# Autodesk Inventor assembly: Front Panel Assembly
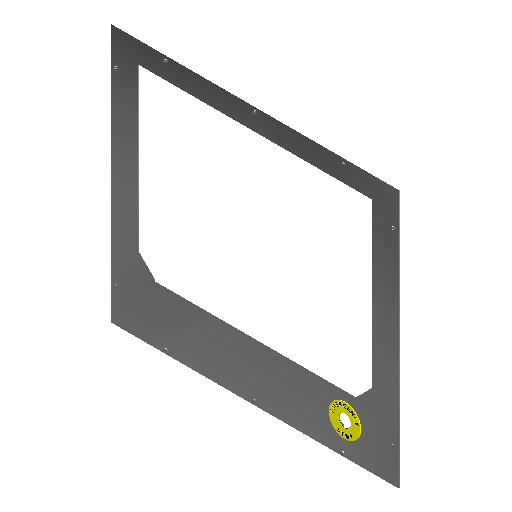
[picture p0: Inventor's stored thumbnail of the model, 512x512]
Saved by Autodesk Inventor 2023.2 (Build 272271000, 271)
## iProperties
Created: 2023-02-06
Part Number: Front Panel Assembly
Document SubType Name: Assembly
Designer: remop
Author: remop
## Documents named in this file (5)
- C:\Users\remop\OneDrive\Documents\Inventor\3D Printers\LuEVO\Mk5_FullKinematic\Front Panel Assembly.iam
- C:\Users\remop\OneDrive\Documents\Inventor\3D Printers\LuEVO\Mk5_FullKinematic\Front Panel.ipt
- C:\Users\remop\OneDrive\Documents\Inventor\Content Center Files\R2023\en-US\AS 1420\AS 1420 - 1973 - M3 x 6.ipt
- C:\Users\remop\OneDrive\Documents\Inventor\3D Printers\LuEVO\Mk5_FullKinematic\E-Stop Plate (Yellow).ipt
- C:\Users\remop\OneDrive\Documents\Inventor\3D Printers\LuEVO\Mk5_FullKinematic\E-Stop Plate (Black).ipt
## Components (13 placed, 4 different names)
1. Front Panel:1 — Insert:1, Insert:2, Insert:3, Insert:4, Insert:5, Insert:6, Insert:7, Insert:8, Insert:9, Insert:10, Rigid:1, Rotational:1
2. AS 1420 - Metric M3 x 6:1 — Insert:1
3. AS 1420 - Metric M3 x 6:2 — Insert:2
4. AS 1420 - Metric M3 x 6:3 — Insert:3
5. AS 1420 - Metric M3 x 6:4 — Insert:4
6. AS 1420 - Metric M3 x 6:5 — Insert:5
7. AS 1420 - Metric M3 x 6:6 — Insert:6
8. AS 1420 - Metric M3 x 6:7 — Insert:7
9. AS 1420 - Metric M3 x 6:8 — Insert:8
10. AS 1420 - Metric M3 x 6:9 — Insert:9
11. AS 1420 - Metric M3 x 6:10 — Insert:10
12. E-Stop Plate (Yellow):1 — Rotational:1
13. E-Stop Plate (Black):1 — Rigid:1
## Relationships (12: Insert 10, WeldJoint 1, RevoluteJoint 1)
- Insert:1: Front Panel:1 ↔ AS 1420 - Metric M3 x 6:1
- Insert:2: Front Panel:1 ↔ AS 1420 - Metric M3 x 6:2
- Insert:3: Front Panel:1 ↔ AS 1420 - Metric M3 x 6:3
- Insert:4: Front Panel:1 ↔ AS 1420 - Metric M3 x 6:4
- Insert:5: Front Panel:1 ↔ AS 1420 - Metric M3 x 6:5
- Insert:6: Front Panel:1 ↔ AS 1420 - Metric M3 x 6:6
- Insert:7: Front Panel:1 ↔ AS 1420 - Metric M3 x 6:7
- Insert:8: Front Panel:1 ↔ AS 1420 - Metric M3 x 6:8
- Insert:9: Front Panel:1 ↔ AS 1420 - Metric M3 x 6:9
- Insert:10: Front Panel:1 ↔ AS 1420 - Metric M3 x 6:10
- Rigid:1 [WeldJoint]: Front Panel:1 ↔ E-Stop Plate (Black):1
- Rotational:1 [RevoluteJoint]: Front Panel:1 ↔ E-Stop Plate (Yellow):1
